# Autodesk Inventor assembly: Base-Rotation
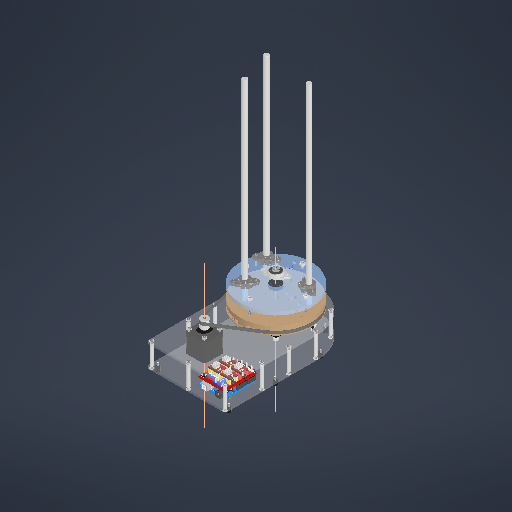
[picture p0: Inventor's stored thumbnail of the model, 512x512]
Saved by Autodesk Inventor 2025.2 (Build 292293000, 293)
## iProperties
Created: 2025-04-10
Part Number: Base-Rotation
Document SubType Name: Assembly
Designer: Tiago
Author: Tiago
## Documents named in this file (26)
- C:\Users\Tiago\Documents\Inventor\Exp. Braço v1\Base-Rotation.iam
- C:\Users\Tiago\Documents\Inventor\Exp. Braço v1\NEMA17 42-38.ipt
- C:\Users\Tiago\Documents\Inventor\Exp. Braço v1\Plataforma_giratoria_4p.iam
- C:\Users\Tiago\Documents\Inventor\Exp. Braço v1\SupBase.ipt
- C:\Users\Tiago\Documents\Inventor\Exp. Braço v1\skf_bearing_608-2z_2.iam
- C:\Users\Tiago\Documents\Inventor\Exp. Braço v1\Linear_Shaft_Support_SHF10.ipt
- C:\Users\Tiago\Documents\Inventor\Exp. Braço v1\rodshaft_10x400.ipt
- C:\Users\Tiago\Documents\Inventor\Exp. Braço v1\Base_solida.ipt
- C:\Users\Tiago\Documents\Inventor\Exp. Braço v1\Arduino_CNC_Assembly.iam
- C:\Users\Tiago\Documents\Inventor\Exp. Braço v1\Base_solida_Down.ipt
- C:\Users\Tiago\Documents\Inventor\Exp. Braço v1\Amortecedor_Borracha.ipt
- C:\Users\Tiago\Documents\Inventor\Exp. Braço v1\Espaçador_m3_L3.5.ipt
- C:\Users\Tiago\Documents\Inventor\Exp. Braço v1\espaçador_M3_L40.ipt
- C:\Users\Tiago\Documents\Inventor\Exp. Braço v1\GT2Pulley_z220.ipt
- GT2Pulley_z220.ipt
- C:\Users\Tiago\Documents\Inventor\Exp. Braço v1\GT2Pulley_z20.ipt
- C:\Users\Tiago\Documents\Inventor\Exp. Braço v1\Base-Rotation\Design Accelerator\Synchronous Belts Transmission3.iam
- C:\Users\Tiago\Documents\Inventor\Exp. Braço v1\Limit_Switch_L1.ipt
- C:\Users\Tiago\Documents\Inventor\Exp. Braço v1\Anilha_M3.ipt
- C:\Users\Tiago\Documents\Inventor\Exp. Braço v1\M3 x0.5 ALT (...).ipt
- C:\Users\Tiago\Documents\Inventor\Exp. Braço v1\M4 x0.7 ALT (...)_L11.ipt
- C:\Users\Tiago\Documents\Inventor\Exp. Braço v1\Porca_sextavada(4M).ipt
- C:\Users\Tiago\Documents\Inventor\Exp. Braço v1\M4 x0.7 ALT (...)_L22.ipt
- C:\Users\Tiago\Documents\Inventor\Exp. Braço v1\M4 x0.7 ALT (...)_L18.ipt
- C:\Users\Tiago\Documents\Inventor\Exp. Braço v1\M5 x0.8ALT (...)_L11.ipt
- C:\Users\Tiago\Documents\Inventor\Exp. Braço v1\KFL08 - Mancal Flange oval Ø8.ipt
## Components (123 placed, 24 different names)
1. NEMA17 42-38:1 — Mate:85, Mate:86, Flush:4, Mate:87, Flush:8
2. Plataforma_giratoria_4p:1 [sub-assembly] — Mate:27, Mate:28, Mate:29, Mate:88, Mate:89, Limit switch, Mate:105, Insert:53, Insert:54, Insert:55, Insert:56, Insert:57, Insert:58, Insert:59, Insert:60
3. SupBase:1 — Mate:9, Mate:11, Mate:12, Mate:13, Mate:14, Mate:15, Mate:16, Mate:17, Mate:18, Mate:19, Mate:91, Mate:93, Flush:5, Mate:94, Mate:105, Mate:123, Mate:125, Mate:128, Mate:129
4. skf_bearing_608-2z_2:1 [sub-assembly] — Mate:9, Flush:5
5. Linear_Shaft_Support_SHF10:1 — Mate:11, Mate:15, Mate:18, Mate:20, Insert:63, Insert:64, Insert:67
6. Linear_Shaft_Support_SHF10:2 — Mate:12, Mate:16, Mate:19, Mate:21, Insert:65, Insert:66, Insert:69
7. Linear_Shaft_Support_SHF10:3 — Mate:13, Mate:14, Mate:17, Mate:22, Insert:61, Insert:62, Insert:68
8. rodshaft_10x400:1 — Mate:22, Mate:100
9. rodshaft_10x400:2 — Mate:21, Mate:101
10. rodshaft_10x400:3 — Mate:20, Mate:99
11. Base_solida:1 — Mate:27, Mate:28, Mate:29, Mate:31, Flush:1, Flush:2, Mate:85, Mate:87, Mate:97, Mate:98, Flush:8, Mate:102, Mate:103, Mate:104, Insert:1, Insert:4, Insert:7, Insert:8, Insert:10, Insert:12, Insert:14, Insert:16, Insert:18, Insert:20, Insert:22, Insert:24, Mate:106, Mate:107, Mate:108, Mate:109, Mate:110, Mate:111, Mate:112, Mate:113, Mate:115, Mate:117, Mate:119, Mate:121
12. Arduino_CNC_Assembly:1 [sub-assembly] — Mate:32, Mate:33, Mate:34, Mate:35, Mate:36
13. Base_solida_Down:1 — Mate:31, Flush:1, Flush:2, Mate:32, Mate:33, Mate:34, Mate:35, Mate:36, Mate:37, Mate:38, Mate:39, Mate:40, Mate:41, Mate:42, Mate:43, Mate:44, Mate:45, Mate:46, Mate:47, Mate:48, Mate:49, Mate:50, Mate:51, Mate:52, Mate:53, Mate:54, Mate:55, Mate:56, Mate:57, Mate:58, Mate:59, Mate:60, Mate:61, Mate:62, Mate:63, Mate:64, Mate:65, Mate:66, Mate:67, Mate:68, Mate:69, Mate:70, Mate:71, Mate:72, Mate:73, Mate:74, Mate:75, Mate:76, Mate:77, Mate:78, Mate:79, Mate:80, Mate:81, Mate:82, Mate:83, Mate:84, Flush:7, Insert:26, Insert:28, Insert:30, Insert:32, Insert:34, Insert:36, Insert:38, Insert:40, Insert:42, Insert:44, Insert:46, Insert:48
14. Amortecedor_Borracha:1 — Mate:50, Mate:57
15. Amortecedor_Borracha:2 — Mate:49, Mate:58
16. Amortecedor_Borracha:3 — Mate:48, Mate:59
17. Amortecedor_Borracha:4 — Mate:51, Mate:56
18. Amortecedor_Borracha:5 — Mate:47, Mate:60
19. Amortecedor_Borracha:6 — Mate:53, Mate:54
20. Amortecedor_Borracha:7 — Mate:45, Mate:46
21. Amortecedor_Borracha:8 — Mate:52, Mate:55
22. Espaçador_m3_L3.5:1 — Mate:37, Mate:41
23. Espaçador_m3_L3.5:2 — Mate:38, Mate:44
24. Espaçador_m3_L3.5:3 — Mate:40, Mate:42
25. Espaçador_m3_L3.5:4 — Mate:39, Mate:43
26. espaçador_M3_L40:1 — Mate:61, Mate:73
27. espaçador_M3_L40:2 — Mate:62, Mate:75
28. espaçador_M3_L40:3 — Mate:63, Mate:76
29. espaçador_M3_L40:4 — Mate:64, Mate:77
30. espaçador_M3_L40:5 — Mate:65, Mate:78
31. espaçador_M3_L40:6 — Mate:66, Mate:79
32. espaçador_M3_L40:7 — Mate:67, Mate:74
33. espaçador_M3_L40:8 — Mate:68, Mate:84
34. espaçador_M3_L40:9 — Mate:69, Mate:83
35. espaçador_M3_L40:10 — Mate:70, Mate:82
36. espaçador_M3_L40:11 — Mate:71, Mate:81
37. espaçador_M3_L40:12 — Mate:72, Mate:80
38. GT2Pulley_z220:1 — Mate:88, Mate:89, Rotação das polias da base(11:1), Limit switch, Mate:93, Mate:94, Mate:95, Mate:99, Mate:100, Mate:101, Mate:130, Mate:131
39. GT2Pulley_z20:1 — Mate:86, Flush:4, Rotação das polias da base(11:1), Mate:96, Flush:6
40. Synchronous Belts Transmission:1 [sub-assembly] — Mate:91, Mate:95, Mate:96, Flush:6
41. Limit_Switch_L1:1 — Mate:102, Mate:103, Mate:104
42. Anilha_M3:1 — Insert:1, Insert:2
43. M3 x0.5 ALT (...):1 — Insert:2
44. Anilha_M3:2 — Insert:4
45. M3 x0.5 ALT (...):2
46. Anilha_M3:3 — Insert:7
47. M3 x0.5 ALT (...):3
48. Anilha_M3:4 — Insert:8
49. M3 x0.5 ALT (...):4
50. Anilha_M3:5 — Insert:10
51. M3 x0.5 ALT (...):5
52. Anilha_M3:6 — Insert:12
53. M3 x0.5 ALT (...):6
54. Anilha_M3:7 — Insert:14
55. M3 x0.5 ALT (...):7
56. Anilha_M3:8 — Insert:16
57. M3 x0.5 ALT (...):8
58. Anilha_M3:9 — Insert:18
59. M3 x0.5 ALT (...):9
60. Anilha_M3:10 — Insert:20
61. M3 x0.5 ALT (...):10
62. Anilha_M3:11 — Insert:22
63. M3 x0.5 ALT (...):11
64. Anilha_M3:12 — Insert:24
65. M3 x0.5 ALT (...):12
66. Anilha_M3:13 — Insert:26
67. M3 x0.5 ALT (...):13
68. Anilha_M3:14 — Insert:28
69. M3 x0.5 ALT (...):14
70. Anilha_M3:15 — Insert:30
71. M3 x0.5 ALT (...):15
72. Anilha_M3:16 — Insert:32
73. M3 x0.5 ALT (...):16
74. Anilha_M3:17 — Insert:34
75. M3 x0.5 ALT (...):17
76. Anilha_M3:18 — Insert:36
77. M3 x0.5 ALT (...):18
78. Anilha_M3:19 — Insert:38
79. M3 x0.5 ALT (...):19
80. Anilha_M3:20 — Insert:40
81. M3 x0.5 ALT (...):20
82. Anilha_M3:21 — Insert:42
83. M3 x0.5 ALT (...):21
84. Anilha_M3:22 — Insert:44
85. M3 x0.5 ALT (...):22
86. Anilha_M3:23 — Insert:46
87. M3 x0.5 ALT (...):23
88. Anilha_M3:24 — Insert:48
89. M3 x0.5 ALT (...):24
90. Anilha_M3:25 — Mate:107
91. M3 x0.5 ALT (...):25 — Mate:106
92. Anilha_M3:26 — Mate:113
93. M3 x0.5 ALT (...):26 — Mate:108
94. Anilha_M3:27 — Mate:112
95. M3 x0.5 ALT (...):27 — Mate:109
96. Anilha_M3:28 — Mate:111
97. M3 x0.5 ALT (...):28 — Mate:110
98. M4 x0.7 ALT (...)_L11:1 — Insert:53, Mate:114
99. Porca_sextavada(4M):1 — Mate:114, Mate:115
100. M4 x0.7 ALT (...)_L11:2 — Insert:54
101. Porca_sextavada(4M):2 — Mate:117
102. M4 x0.7 ALT (...)_L11:3 — Insert:55
103. Porca_sextavada(4M):3 — Mate:119
104. M4 x0.7 ALT (...)_L11:4 — Insert:56
105. Porca_sextavada(4M):4 — Mate:121
106. M4 x0.7 ALT (...)_L22:1 — Insert:57, Mate:122
107. Porca_sextavada(4M):5 — Mate:122, Mate:123
108. M4 x0.7 ALT (...)_L22:5 — Insert:58
109. Porca_sextavada(4M):6 — Mate:125
110. M4 x0.7 ALT (...)_L22:6 — Insert:59
111. Porca_sextavada(4M):7 — Mate:129
112. M4 x0.7 ALT (...)_L22:7 — Insert:60
113. Porca_sextavada(4M):8 — Mate:128
114. M4 x0.7 ALT (...)_L18:1 — Insert:61
115. M4 x0.7 ALT (...)_L11:5 — Insert:62
116. M4 x0.7 ALT (...)_L11:6 — Insert:64
117. M4 x0.7 ALT (...)_L11:7 — Insert:63
118. M4 x0.7 ALT (...)_L11:8 — Insert:65
119. M4 x0.7 ALT (...)_L11:9 — Insert:66
120. M5 x0.8ALT (...)_L11:1 — Insert:67
121. M5 x0.8ALT (...)_L11:2 — Insert:68
122. M5 x0.8ALT (...)_L11:3 — Insert:69
123. KFL08 - Mancal Flange oval Ø8:1 — Mate:130, Mate:131
## Relationships (193: Mate 115, Insert 69, Flush 7, RelateRotation 1, Angle 1)
- Mate:9: SupBase:1 ↔ skf_bearing_608-2z_2:1
- Mate:11: SupBase:1 ↔ Linear_Shaft_Support_SHF10:1
- Mate:12: SupBase:1 ↔ Linear_Shaft_Support_SHF10:2
- Mate:13: SupBase:1 ↔ Linear_Shaft_Support_SHF10:3
- Mate:14: SupBase:1 ↔ Linear_Shaft_Support_SHF10:3
- Mate:15: SupBase:1 ↔ Linear_Shaft_Support_SHF10:1
- Mate:16: SupBase:1 ↔ Linear_Shaft_Support_SHF10:2
- Mate:17: SupBase:1 ↔ Linear_Shaft_Support_SHF10:3
- Mate:18: SupBase:1 ↔ Linear_Shaft_Support_SHF10:1
- Mate:19: SupBase:1 ↔ Linear_Shaft_Support_SHF10:2
- Mate:20: Linear_Shaft_Support_SHF10:1 ↔ rodshaft_10x400:3
- Mate:21: Linear_Shaft_Support_SHF10:2 ↔ rodshaft_10x400:2
- Mate:22: Linear_Shaft_Support_SHF10:3 ↔ rodshaft_10x400:1
- Mate:27: Plataforma_giratoria_4p:1 ↔ Base_solida:1
- Mate:28: Plataforma_giratoria_4p:1 ↔ Base_solida:1
- Mate:29: Plataforma_giratoria_4p:1 ↔ Base_solida:1
- Mate:31 (40 mm): Base_solida:1 ↔ Base_solida_Down:1
- Flush:1: Base_solida:1 ↔ Base_solida_Down:1
- Flush:2: Base_solida:1 ↔ Base_solida_Down:1
- Mate:32 (3.5 mm): Arduino_CNC_Assembly:1 ↔ Base_solida_Down:1
- Mate:33: Arduino_CNC_Assembly:1 ↔ Base_solida_Down:1
- Mate:34: Arduino_CNC_Assembly:1 ↔ Base_solida_Down:1
- Mate:35: Arduino_CNC_Assembly:1 ↔ Base_solida_Down:1
- Mate:36: Arduino_CNC_Assembly:1 ↔ Base_solida_Down:1
- Mate:37: Base_solida_Down:1 ↔ Espaçador_m3_L3.5:1
- Mate:38: Base_solida_Down:1 ↔ Espaçador_m3_L3.5:2
- Mate:39: Base_solida_Down:1 ↔ Espaçador_m3_L3.5:4
- Mate:40: Base_solida_Down:1 ↔ Espaçador_m3_L3.5:3
- Mate:41: Base_solida_Down:1 ↔ Espaçador_m3_L3.5:1
- Mate:42: Base_solida_Down:1 ↔ Espaçador_m3_L3.5:3
- Mate:43: Base_solida_Down:1 ↔ Espaçador_m3_L3.5:4
- Mate:44: Base_solida_Down:1 ↔ Espaçador_m3_L3.5:2
- Mate:45: Base_solida_Down:1 ↔ Amortecedor_Borracha:7
- Mate:46: Base_solida_Down:1 ↔ Amortecedor_Borracha:7
- Mate:47: Base_solida_Down:1 ↔ Amortecedor_Borracha:5
- Mate:48: Base_solida_Down:1 ↔ Amortecedor_Borracha:3
- Mate:49: Base_solida_Down:1 ↔ Amortecedor_Borracha:2
- Mate:50: Base_solida_Down:1 ↔ Amortecedor_Borracha:1
- Mate:51: Base_solida_Down:1 ↔ Amortecedor_Borracha:4
- Mate:52: Base_solida_Down:1 ↔ Amortecedor_Borracha:8
- Mate:53: Base_solida_Down:1 ↔ Amortecedor_Borracha:6
- Mate:54: Base_solida_Down:1 ↔ Amortecedor_Borracha:6
- Mate:55: Base_solida_Down:1 ↔ Amortecedor_Borracha:8
- Mate:56: Base_solida_Down:1 ↔ Amortecedor_Borracha:4
- Mate:57: Base_solida_Down:1 ↔ Amortecedor_Borracha:1
- Mate:58: Base_solida_Down:1 ↔ Amortecedor_Borracha:2
- Mate:59: Base_solida_Down:1 ↔ Amortecedor_Borracha:3
- Mate:60: Base_solida_Down:1 ↔ Amortecedor_Borracha:5
- Mate:61: Base_solida_Down:1 ↔ espaçador_M3_L40:1
- Mate:62: Base_solida_Down:1 ↔ espaçador_M3_L40:2
- Mate:63: Base_solida_Down:1 ↔ espaçador_M3_L40:3
- Mate:64: Base_solida_Down:1 ↔ espaçador_M3_L40:4
- Mate:65: Base_solida_Down:1 ↔ espaçador_M3_L40:5
- Mate:66: Base_solida_Down:1 ↔ espaçador_M3_L40:6
- Mate:67: Base_solida_Down:1 ↔ espaçador_M3_L40:7
- Mate:68: Base_solida_Down:1 ↔ espaçador_M3_L40:8
- Mate:69: Base_solida_Down:1 ↔ espaçador_M3_L40:9
- Mate:70: Base_solida_Down:1 ↔ espaçador_M3_L40:10
- Mate:71: Base_solida_Down:1 ↔ espaçador_M3_L40:11
- Mate:72: Base_solida_Down:1 ↔ espaçador_M3_L40:12
- Mate:73: Base_solida_Down:1 ↔ espaçador_M3_L40:1
- Mate:74: Base_solida_Down:1 ↔ espaçador_M3_L40:7
- Mate:75: Base_solida_Down:1 ↔ espaçador_M3_L40:2
- Mate:76: Base_solida_Down:1 ↔ espaçador_M3_L40:3
- Mate:77: Base_solida_Down:1 ↔ espaçador_M3_L40:4
- Mate:78: Base_solida_Down:1 ↔ espaçador_M3_L40:5
- Mate:79: Base_solida_Down:1 ↔ espaçador_M3_L40:6
- Mate:80: Base_solida_Down:1 ↔ espaçador_M3_L40:12
- Mate:81: Base_solida_Down:1 ↔ espaçador_M3_L40:11
- Mate:82: Base_solida_Down:1 ↔ espaçador_M3_L40:10
- Mate:83: Base_solida_Down:1 ↔ espaçador_M3_L40:9
- Mate:84: Base_solida_Down:1 ↔ espaçador_M3_L40:8
- Mate:85: NEMA17 42-38:1 ↔ Base_solida:1
- Mate:86: NEMA17 42-38:1 ↔ GT2Pulley_z20:1
- Flush:4 (-0.8 mm): NEMA17 42-38:1 ↔ GT2Pulley_z20:1
- Mate:87: NEMA17 42-38:1 ↔ Base_solida:1
- Mate:88: Plataforma_giratoria_4p:1 ↔ GT2Pulley_z220:1
- Mate:89: Plataforma_giratoria_4p:1 ↔ GT2Pulley_z220:1
- Rotação das polias da base(11:1) [RelateRotation] (11 ul): GT2Pulley_z220:1 ↔ GT2Pulley_z20:1
- Limit switch [Angle] (0 deg): Plataforma_giratoria_4p:1 ↔ GT2Pulley_z220:1
- Mate:91: SupBase:1 ↔ Synchronous Belts Transmission:1
- Mate:93: SupBase:1 ↔ GT2Pulley_z220:1
- Flush:5: SupBase:1 ↔ skf_bearing_608-2z_2:1
- Mate:94: SupBase:1 ↔ GT2Pulley_z220:1
- Mate:95: GT2Pulley_z220:1 ↔ Synchronous Belts Transmission:1
- Mate:96: GT2Pulley_z20:1 ↔ Synchronous Belts Transmission:1
- Flush:6 (2 mm): GT2Pulley_z20:1 ↔ Synchronous Belts Transmission:1
- Flush:7: Base_solida_Down:1
- Mate:97: Base_solida:1
- Mate:98: Base_solida:1
- Mate:99: rodshaft_10x400:3 ↔ GT2Pulley_z220:1
- Mate:100: rodshaft_10x400:1 ↔ GT2Pulley_z220:1
- Mate:101: rodshaft_10x400:2 ↔ GT2Pulley_z220:1
- Flush:8 (59.286 mm): NEMA17 42-38:1 ↔ Base_solida:1
- Mate:102: Base_solida:1 ↔ Limit_Switch_L1:1
- Mate:103: Base_solida:1 ↔ Limit_Switch_L1:1
- Mate:104: Base_solida:1 ↔ Limit_Switch_L1:1
- Insert:1: Base_solida:1 ↔ Anilha_M3:1
- Insert:2: Anilha_M3:1 ↔ M3 x0.5 ALT (...):1
- [Insert]: Anilha_M3:2 ↔ M3 x0.5 ALT (...):2
- Insert:4: Base_solida:1 ↔ Anilha_M3:2
- [Insert]: Anilha_M3:3 ↔ M3 x0.5 ALT (...):3
- [Insert]: Anilha_M3:4 ↔ M3 x0.5 ALT (...):4
- Insert:7: Base_solida:1 ↔ Anilha_M3:3
- Insert:8: Base_solida:1 ↔ Anilha_M3:4
- [Insert]: Anilha_M3:5 ↔ M3 x0.5 ALT (...):5
- Insert:10: Base_solida:1 ↔ Anilha_M3:5
- [Insert]: Anilha_M3:6 ↔ M3 x0.5 ALT (...):6
- Insert:12: Base_solida:1 ↔ Anilha_M3:6
- [Insert]: Anilha_M3:7 ↔ M3 x0.5 ALT (...):7
- Insert:14: Base_solida:1 ↔ Anilha_M3:7
- [Insert]: Anilha_M3:8 ↔ M3 x0.5 ALT (...):8
- Insert:16: Base_solida:1 ↔ Anilha_M3:8
- [Insert]: Anilha_M3:9 ↔ M3 x0.5 ALT (...):9
- Insert:18: Base_solida:1 ↔ Anilha_M3:9
- [Insert]: Anilha_M3:10 ↔ M3 x0.5 ALT (...):10
- Insert:20: Base_solida:1 ↔ Anilha_M3:10
- [Insert]: Anilha_M3:11 ↔ M3 x0.5 ALT (...):11
- Insert:22: Base_solida:1 ↔ Anilha_M3:11
- [Insert]: Anilha_M3:12 ↔ M3 x0.5 ALT (...):12
- Insert:24: Base_solida:1 ↔ Anilha_M3:12
- [Insert]: Anilha_M3:13 ↔ M3 x0.5 ALT (...):13
- Insert:26: Base_solida_Down:1 ↔ Anilha_M3:13
- [Insert]: Anilha_M3:14 ↔ M3 x0.5 ALT (...):14
- Insert:28: Base_solida_Down:1 ↔ Anilha_M3:14
- [Insert]: Anilha_M3:15 ↔ M3 x0.5 ALT (...):15
- Insert:30: Base_solida_Down:1 ↔ Anilha_M3:15
- [Insert]: Anilha_M3:16 ↔ M3 x0.5 ALT (...):16
- Insert:32: Base_solida_Down:1 ↔ Anilha_M3:16
- [Insert]: Anilha_M3:17 ↔ M3 x0.5 ALT (...):17
- Insert:34: Base_solida_Down:1 ↔ Anilha_M3:17
- [Insert]: Anilha_M3:18 ↔ M3 x0.5 ALT (...):18
- Insert:36: Base_solida_Down:1 ↔ Anilha_M3:18
- [Insert]: Anilha_M3:19 ↔ M3 x0.5 ALT (...):19
- Insert:38: Base_solida_Down:1 ↔ Anilha_M3:19
- [Insert]: Anilha_M3:20 ↔ M3 x0.5 ALT (...):20
- Insert:40: Base_solida_Down:1 ↔ Anilha_M3:20
- [Insert]: Anilha_M3:21 ↔ M3 x0.5 ALT (...):21
- Insert:42: Base_solida_Down:1 ↔ Anilha_M3:21
- [Insert]: Anilha_M3:22 ↔ M3 x0.5 ALT (...):22
- Insert:44: Base_solida_Down:1 ↔ Anilha_M3:22
- [Insert]: Anilha_M3:23 ↔ M3 x0.5 ALT (...):23
- Insert:46: Base_solida_Down:1 ↔ Anilha_M3:23
- [Insert]: Anilha_M3:24 ↔ M3 x0.5 ALT (...):24
- Insert:48: Base_solida_Down:1 ↔ Anilha_M3:24
- Mate:105: Plataforma_giratoria_4p:1 ↔ SupBase:1
- [Insert]: Anilha_M3:25 ↔ M3 x0.5 ALT (...):25
- Mate:106: Base_solida:1 ↔ M3 x0.5 ALT (...):25
- Mate:107: Base_solida:1 ↔ Anilha_M3:25
- [Insert]: Anilha_M3:26 ↔ M3 x0.5 ALT (...):26
- [Insert]: Anilha_M3:27 ↔ M3 x0.5 ALT (...):27
- [Insert]: Anilha_M3:28 ↔ M3 x0.5 ALT (...):28
- Mate:108: Base_solida:1 ↔ M3 x0.5 ALT (...):26
- Mate:109: Base_solida:1 ↔ M3 x0.5 ALT (...):27
- Mate:110: Base_solida:1 ↔ M3 x0.5 ALT (...):28
- Mate:111: Base_solida:1 ↔ Anilha_M3:28
- Mate:112: Base_solida:1 ↔ Anilha_M3:27
- Mate:113: Base_solida:1 ↔ Anilha_M3:26
- Insert:53: Plataforma_giratoria_4p:1 ↔ M4 x0.7 ALT (...)_L11:1
- Mate:114: M4 x0.7 ALT (...)_L11:1 ↔ Porca_sextavada(4M):1
- Mate:115: Base_solida:1 ↔ Porca_sextavada(4M):1
- [Mate]: M4 x0.7 ALT (...)_L11:2 ↔ Porca_sextavada(4M):2
- Insert:54: Plataforma_giratoria_4p:1 ↔ M4 x0.7 ALT (...)_L11:2
- Mate:117: Base_solida:1 ↔ Porca_sextavada(4M):2
- [Mate]: M4 x0.7 ALT (...)_L11:3 ↔ Porca_sextavada(4M):3
- Insert:55: Plataforma_giratoria_4p:1 ↔ M4 x0.7 ALT (...)_L11:3
- Mate:119: Base_solida:1 ↔ Porca_sextavada(4M):3
- [Mate]: M4 x0.7 ALT (...)_L11:4 ↔ Porca_sextavada(4M):4
- Insert:56: Plataforma_giratoria_4p:1 ↔ M4 x0.7 ALT (...)_L11:4
- Mate:121: Base_solida:1 ↔ Porca_sextavada(4M):4
- Insert:57: Plataforma_giratoria_4p:1 ↔ M4 x0.7 ALT (...)_L22:1
- Mate:122: M4 x0.7 ALT (...)_L22:1 ↔ Porca_sextavada(4M):5
- Mate:123: SupBase:1 ↔ Porca_sextavada(4M):5
- [Mate]: M4 x0.7 ALT (...)_L22:5 ↔ Porca_sextavada(4M):6
- Insert:58: Plataforma_giratoria_4p:1 ↔ M4 x0.7 ALT (...)_L22:5
- Mate:125: SupBase:1 ↔ Porca_sextavada(4M):6
- [Mate]: M4 x0.7 ALT (...)_L22:6 ↔ Porca_sextavada(4M):7
- Insert:59: Plataforma_giratoria_4p:1 ↔ M4 x0.7 ALT (...)_L22:6
- [Mate]: M4 x0.7 ALT (...)_L22:7 ↔ Porca_sextavada(4M):8
- Insert:60: Plataforma_giratoria_4p:1 ↔ M4 x0.7 ALT (...)_L22:7
- Mate:128: SupBase:1 ↔ Porca_sextavada(4M):8
- Mate:129: SupBase:1 ↔ Porca_sextavada(4M):7
- Insert:61: Linear_Shaft_Support_SHF10:3 ↔ M4 x0.7 ALT (...)_L18:1
- Insert:62: Linear_Shaft_Support_SHF10:3 ↔ M4 x0.7 ALT (...)_L11:5
- Insert:63: Linear_Shaft_Support_SHF10:1 ↔ M4 x0.7 ALT (...)_L11:7
- Insert:64: Linear_Shaft_Support_SHF10:1 ↔ M4 x0.7 ALT (...)_L11:6
- Insert:65: Linear_Shaft_Support_SHF10:2 ↔ M4 x0.7 ALT (...)_L11:8
- Insert:66: Linear_Shaft_Support_SHF10:2 ↔ M4 x0.7 ALT (...)_L11:9
- Insert:67: Linear_Shaft_Support_SHF10:1 ↔ M5 x0.8ALT (...)_L11:1
- Insert:68: Linear_Shaft_Support_SHF10:3 ↔ M5 x0.8ALT (...)_L11:2
- Insert:69: Linear_Shaft_Support_SHF10:2 ↔ M5 x0.8ALT (...)_L11:3
- Mate:130: GT2Pulley_z220:1 ↔ KFL08 - Mancal Flange oval Ø8:1
- Mate:131: GT2Pulley_z220:1 ↔ KFL08 - Mancal Flange oval Ø8:1
## Named parameters: d204_d203 = 0 mm, d206_d204_d203 = 0 mm, d207_d204_d203 = 0 mm, d210_d204_d203 = 0 mm, d212_d204_d203 = 0 mm, d214_d204_d203 = 0 mm, d216_d204_d203 = 0 mm, d218_d204_d203 = 0 mm, d220_d204_d203 = 0 mm, d222_d204_d203 = 0 mm, d224_d204_d203 = 0 mm, d226_d204_d203 = 0 mm, d228_d204_d203 = 0 mm, d230_d204_d203 = 0 mm, d232_d204_d203 = 0 mm, d234_d204_d203 = 0 mm, d236_d204_d203 = 0 mm, d238_d204_d203 = 0 mm, d240_d204_d203 = 0 mm, d242_d204_d203 = 0 mm, d244_d204_d203 = 0 mm, d246_d204_d203 = 0 mm, d248_d204_d203 = 0 mm, d251_d216_d204_d203 = 0 mm, d254_d216_d204_d203 = 0 mm, d255_d216_d204_d203 = 0 mm, d256_d216_d204_d203 = 0 mm, d266_d264 = 0 mm, d269_d264 = 0 mm, d272_d264 = 0 mm, d280_d278 = 0 mm, d283_d278 = 0 mm, d285_d278 = 0 mm
